# Autodesk Inventor assembly: Hooded Shooter MASTER
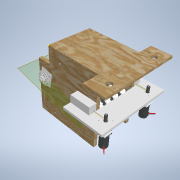
[picture p0: Inventor's stored thumbnail of the model, 180x180]
Saved by Autodesk Inventor 2020 (Build 240168000, 168)
## iProperties
Created: 2020-01-13
Part Number: Hooded Shooter MASTER
Document SubType Name: Assembly
Designer: autum
Author: autum
## Documents named in this file (17)
- D:\Users\JimAndVal\Documents\JIM\IronRiders\2020 Robot-1\Manipulators\Hooded Shooter (Protected Zone)\Hooded Shooter MASTER.iam
- D:\Users\JimAndVal\Documents\JIM\IronRiders\2020 Robot-1\Manipulators\Hooded Shooter (Protected Zone)\Hood.ipt
- D:\Users\JimAndVal\Documents\JIM\IronRiders\2020 Robot-1\Manipulators\Hooded Shooter (Protected Zone)\Hex Bearing.ipt
- D:\Users\JimAndVal\Documents\JIM\IronRiders\2020 Robot-1\Manipulators\Hooded Shooter (Protected Zone)\Hex Shaft.ipt
- D:\Users\JimAndVal\Documents\JIM\IronRiders\2020 Robot-1\Manipulators\Hooded Shooter (Protected Zone)\Hood (inside).ipt
- D:\Users\JimAndVal\Documents\JIM\IronRiders\2020 Robot-1\Manipulators\Hooded Shooter (Protected Zone)\Threaded rod.ipt
- D:\Users\JimAndVal\Documents\JIM\IronRiders\2020 Robot-1\Manipulators\Hooded Shooter (Protected Zone)\Shaft Mount with NEO mount.ipt
- D:\Users\JimAndVal\Documents\JIM\IronRiders\2020 Robot-1\Manipulators\Hooded Shooter (Protected Zone)\shooter bottom.ipt
- D:\Users\JimAndVal\Documents\JIM\IronRiders\2020 Robot-1\Manipulators\Hooded Shooter (Protected Zone)\am-2256 4 in HiGrip Wheel.iam
- D:\Users\JimAndVal\Documents\JIM\IronRiders\2020 Robot-1\Manipulators\Hooded Shooter (Protected Zone)\Shooter Base Cleat.ipt
- D:\Users\JimAndVal\Documents\JIM\IronRiders\2020 Robot-1\Manipulators\Hooded Shooter (Protected Zone)\1_5 inch PVC Spacer.ipt
- D:\Users\JimAndVal\Documents\JIM\IronRiders\2020 Robot-1\Manipulators\Hooded Shooter (Protected Zone)\Indexer Upper Plate.ipt
- D:\Users\JimAndVal\Documents\JIM\IronRiders\2020 Robot-1\Indexer 2.0\VersaPlanetary_v2_Single_Stage_10_1_with_BAG.iam
- D:\Users\JimAndVal\Documents\JIM\IronRiders\2020 Robot-1\Manipulators\Hooded Shooter (Protected Zone)\upper indexer plate cleat.ipt
- D:\Users\JimAndVal\Documents\JIM\IronRiders\2020 Robot-1\Manipulators\Hooded Shooter (Protected Zone)\Shooter Motor.iam
- D:\Users\JimAndVal\Documents\JIM\IronRiders\2020 Robot-1\Manipulators\Hooded Shooter (Protected Zone)\_16t_Aluminum_Hub_Sprocket_25_Chain_1_2_Hex_Bore_217-2642.ipt
- D:\Users\JimAndVal\Documents\JIM\IronRiders\2020 Robot-1\Manipulators\Hooded Shooter (Protected Zone)\Clamping_Shaft_Collar_-_1_2_Hex_ID_217-2737(1).ipt
## Components (39 placed, 16 different names)
1. Hood:1 — Mate:34, Flush:7, Mate:37, Mate:38, Mate:73, Mate:75
2. Hood:2 — Mate:35, Flush:6, Mate:40, Mate:72, Mate:74, Mate:79
3. Hex Bearing:1 — Mate:24, Mate:25, Insert:7
4. Hex Bearing:2 — Mate:14, Mate:15, Insert:8
5. Hex Shaft:1 — Mate:14, Mate:15, Mate:24, Mate:25, Flush:8, Mate:42, Mate:43, Mate:44, Mate:45, Mate:46, Mate:47, Mate:48, Mate:49, Mate:94, Flush:22
6. Hood (inside):1 — Mate:34, Mate:35, Flush:6, Flush:7, Mate:39, Mate:41, Mate:55, Mate:57, Mate:59, Mate:61, Mate:64, Mate:65
7. Threaded rod:2 — Mate:58, Mate:60, Mate:70, Mate:71, Mate:78
8. Threaded rod:3 — Mate:62, Mate:63, Mate:68, Mate:69, Mate:80
9. Threaded rod:4 — Mate:54, Mate:56, Mate:66, Mate:67, Mate:76
10. Shaft Mount with NEO mount:1 — Flush:1, Flush:2, Mate:33, Mate:36, Insert:8, Mate:53, Mate:76, Mate:78, Mate:80, Flush:10, Mate:88, Mate:92, Mate:93, Mate:96
11. Shaft Mount with NEO mount:2 — Flush:1, Flush:2, Flush:4, Mate:36, Mate:37, Mate:41, Insert:7, Flush:8, Mate:51, Mate:90
12. shooter bottom:1 — Mate:33, Flush:4, Mate:38, Mate:39, Mate:40, Mate:50, Mate:52, Flush:10, Flush:11, Flush:12, Flush:13, Flush:14, Mate:81
13. am-2256 4 in HiGrip Wheel:1 [sub-assembly] — Mate:42, Mate:43
14. am-2256 4 in HiGrip Wheel:2 [sub-assembly] — Mate:44, Mate:45
15. am-2256 4 in HiGrip Wheel:3 [sub-assembly] — Mate:48, Mate:49
16. am-2256 4 in HiGrip Wheel:4 [sub-assembly] — Mate:46, Mate:47
17. Shooter Base Cleat:1 — Mate:50, Mate:51, Flush:11, Flush:12
18. Shooter Base Cleat:2 — Mate:52, Mate:53
19. 1_5 inch PVC Spacer:1 — Mate:56, Mate:57
20. 1_5 inch PVC Spacer:2 — Mate:54, Mate:55
21. 1_5 inch PVC Spacer:3 — Mate:58, Mate:59
22. 1_5 inch PVC Spacer:4 — Mate:63, Mate:65
23. 1_5 inch PVC Spacer:5 — Mate:62, Mate:64
24. 1_5 inch PVC Spacer:6 — Mate:60, Mate:61
25. 1_5 inch PVC Spacer:7 — Mate:71, Mate:79
26. 1_5 inch PVC Spacer:8 — Mate:70
27. 1_5 inch PVC Spacer:9 — Mate:66, Mate:72
28. 1_5 inch PVC Spacer:10 — Mate:67, Mate:73
29. 1_5 inch PVC Spacer:11 — Mate:68, Mate:74
30. 1_5 inch PVC Spacer:12 — Mate:69, Mate:75
31. Indexer Upper Plate:1 — Flush:13, Flush:14, Mate:81, Mate:82, Mate:83, Mate:84, Flush:15, Flush:16, Mate:86, Mate:87, Angle:1, Flush:17, Mate:89, Flush:18, Mate:91
32. VersaPlanetary_v2_Single_Stage_10_1_with_BAG:1 [sub-assembly] — Mate:82, Mate:83, Mate:84, Mate:85
33. VersaPlanetary_v2_Single_Stage_10_1_with_BAG:2 [sub-assembly] — Mate:86, Mate:87, Angle:1
34. upper indexer plate cleat:1 — Mate:88, Flush:17, Mate:89
35. upper indexer plate cleat:2 — Mate:90, Flush:18, Mate:91
36. Shooter Motor:1 [sub-assembly] — Mate:92, Mate:93, Mate:95, Angle:2
37. _16t_Aluminum_Hub_Sprocket_25_Chain_1_2_Hex_Bore_217-2642:1 — Mate:97, Mate:98, Mate:99, Mate:100
38. Clamping_Shaft_Collar_-_1_2_Hex_ID_217-2737(1):1 — Mate:96, Mate:97, Mate:99, Flush:22
39. Clamping_Shaft_Collar_-_1_2_Hex_ID_217-2737(1):2 — Mate:98, Mate:100
## Relationships (92: Mate 71, Flush 17, Insert 2, Angle 2)
- Mate:14: Hex Bearing:2 ↔ Hex Shaft:1
- Mate:15: Hex Bearing:2 ↔ Hex Shaft:1
- Mate:24: Hex Bearing:1 ↔ Hex Shaft:1
- Mate:25: Hex Bearing:1 ↔ Hex Shaft:1
- Flush:1: Shaft Mount with NEO mount:1 ↔ Shaft Mount with NEO mount:2
- Flush:2: Shaft Mount with NEO mount:1 ↔ Shaft Mount with NEO mount:2
- Mate:33: Shaft Mount with NEO mount:1 ↔ shooter bottom:1
- Flush:4: Shaft Mount with NEO mount:2 ↔ shooter bottom:1
- Mate:34 (38.1 mm): Hood:1 ↔ Hood (inside):1
- Mate:35 (38.1 mm): Hood:2 ↔ Hood (inside):1
- Flush:6: Hood:2 ↔ Hood (inside):1
- Flush:7: Hood:1 ↔ Hood (inside):1
- Mate:36 (190.5 mm): Shaft Mount with NEO mount:1 ↔ Shaft Mount with NEO mount:2
- Mate:37 (38.1 mm): Hood:1 ↔ Shaft Mount with NEO mount:2
- Mate:38: Hood:1 ↔ shooter bottom:1
- Mate:39: Hood (inside):1 ↔ shooter bottom:1
- Mate:40: Hood:2 ↔ shooter bottom:1
- Mate:41: Hood (inside):1 ↔ Shaft Mount with NEO mount:2
- Insert:7: Hex Bearing:1 ↔ Shaft Mount with NEO mount:2
- Insert:8: Hex Bearing:2 ↔ Shaft Mount with NEO mount:1
- Flush:8 (-25.4 mm): Hex Shaft:1 ↔ Shaft Mount with NEO mount:2
- Mate:42: Hex Shaft:1 ↔ am-2256 4 in HiGrip Wheel:1
- Mate:43: Hex Shaft:1 ↔ am-2256 4 in HiGrip Wheel:1
- Mate:44: Hex Shaft:1 ↔ am-2256 4 in HiGrip Wheel:2
- Mate:45: Hex Shaft:1 ↔ am-2256 4 in HiGrip Wheel:2
- Mate:46: Hex Shaft:1 ↔ am-2256 4 in HiGrip Wheel:4
- Mate:47: Hex Shaft:1 ↔ am-2256 4 in HiGrip Wheel:4
- Mate:48: Hex Shaft:1 ↔ am-2256 4 in HiGrip Wheel:3
- Mate:49: Hex Shaft:1 ↔ am-2256 4 in HiGrip Wheel:3
- Mate:50: shooter bottom:1 ↔ Shooter Base Cleat:1
- Mate:51: Shaft Mount with NEO mount:2 ↔ Shooter Base Cleat:1
- Mate:52: shooter bottom:1 ↔ Shooter Base Cleat:2
- Mate:53: Shaft Mount with NEO mount:1 ↔ Shooter Base Cleat:2
- Mate:54: Threaded rod:4 ↔ 1_5 inch PVC Spacer:2
- Mate:55: Hood (inside):1 ↔ 1_5 inch PVC Spacer:2
- Mate:56: Threaded rod:4 ↔ 1_5 inch PVC Spacer:1
- Mate:57: Hood (inside):1 ↔ 1_5 inch PVC Spacer:1
- Mate:58: Threaded rod:2 ↔ 1_5 inch PVC Spacer:3
- Mate:59: Hood (inside):1 ↔ 1_5 inch PVC Spacer:3
- Mate:60: Threaded rod:2 ↔ 1_5 inch PVC Spacer:6
- Mate:61: Hood (inside):1 ↔ 1_5 inch PVC Spacer:6
- Mate:62: Threaded rod:3 ↔ 1_5 inch PVC Spacer:5
- Mate:63: Threaded rod:3 ↔ 1_5 inch PVC Spacer:4
- Mate:64: Hood (inside):1 ↔ 1_5 inch PVC Spacer:5
- Mate:65: Hood (inside):1 ↔ 1_5 inch PVC Spacer:4
- Mate:66: Threaded rod:4 ↔ 1_5 inch PVC Spacer:9
- Mate:67: Threaded rod:4 ↔ 1_5 inch PVC Spacer:10
- Mate:68: Threaded rod:3 ↔ 1_5 inch PVC Spacer:11
- Mate:69: Threaded rod:3 ↔ 1_5 inch PVC Spacer:12
- Mate:70: Threaded rod:2 ↔ 1_5 inch PVC Spacer:8
- Mate:71: Threaded rod:2 ↔ 1_5 inch PVC Spacer:7
- Mate:72: Hood:2 ↔ 1_5 inch PVC Spacer:9
- Mate:73: Hood:1 ↔ 1_5 inch PVC Spacer:10
- Mate:74: Hood:2 ↔ 1_5 inch PVC Spacer:11
- Mate:75: Hood:1 ↔ 1_5 inch PVC Spacer:12
- Mate:76: Threaded rod:4 ↔ Shaft Mount with NEO mount:1
- Mate:78: Threaded rod:2 ↔ Shaft Mount with NEO mount:1
- Mate:79: Hood:2 ↔ 1_5 inch PVC Spacer:7
- Mate:80: Threaded rod:3 ↔ Shaft Mount with NEO mount:1
- Flush:10: Shaft Mount with NEO mount:1 ↔ shooter bottom:1
- Flush:11: shooter bottom:1 ↔ Shooter Base Cleat:1
- Flush:12: shooter bottom:1 ↔ Shooter Base Cleat:1
- Flush:13: shooter bottom:1 ↔ Indexer Upper Plate:1
- Flush:14: shooter bottom:1 ↔ Indexer Upper Plate:1
- Mate:81 (165.1 mm): shooter bottom:1 ↔ Indexer Upper Plate:1
- Mate:82: Indexer Upper Plate:1 ↔ VersaPlanetary_v2_Single_Stage_10_1_with_BAG:1
- Mate:83: Indexer Upper Plate:1 ↔ VersaPlanetary_v2_Single_Stage_10_1_with_BAG:1
- Mate:84: Indexer Upper Plate:1 ↔ VersaPlanetary_v2_Single_Stage_10_1_with_BAG:1
- Flush:15 (-63.5 mm): Indexer Upper Plate:1
- Mate:85: VersaPlanetary_v2_Single_Stage_10_1_with_BAG:1
- Flush:16 (-63.5 mm): Indexer Upper Plate:1
- Mate:86: Indexer Upper Plate:1 ↔ VersaPlanetary_v2_Single_Stage_10_1_with_BAG:2
- Mate:87: Indexer Upper Plate:1 ↔ VersaPlanetary_v2_Single_Stage_10_1_with_BAG:2
- Angle:1 (180 deg): Indexer Upper Plate:1 ↔ VersaPlanetary_v2_Single_Stage_10_1_with_BAG:2
- Mate:88: Shaft Mount with NEO mount:1 ↔ upper indexer plate cleat:1
- Flush:17: Indexer Upper Plate:1 ↔ upper indexer plate cleat:1
- Mate:89: Indexer Upper Plate:1 ↔ upper indexer plate cleat:1
- Mate:90: Shaft Mount with NEO mount:2 ↔ upper indexer plate cleat:2
- Flush:18: Indexer Upper Plate:1 ↔ upper indexer plate cleat:2
- Mate:91: Indexer Upper Plate:1 ↔ upper indexer plate cleat:2
- Flush:21 (17.9578 mm)
- Mate:92: Shaft Mount with NEO mount:1 ↔ Shooter Motor:1
- Mate:93: Shaft Mount with NEO mount:1 ↔ Shooter Motor:1
- Mate:94: Hex Shaft:1
- Mate:95: Shooter Motor:1
- Angle:2 (90 deg): Shooter Motor:1
- Mate:96: Shaft Mount with NEO mount:1 ↔ Clamping_Shaft_Collar_-_1_2_Hex_ID_217-2737(1):1
- Mate:97: _16t_Aluminum_Hub_Sprocket_25_Chain_1_2_Hex_Bore_217-2642:1 ↔ Clamping_Shaft_Collar_-_1_2_Hex_ID_217-2737(1):1
- Mate:98: _16t_Aluminum_Hub_Sprocket_25_Chain_1_2_Hex_Bore_217-2642:1 ↔ Clamping_Shaft_Collar_-_1_2_Hex_ID_217-2737(1):2
- Mate:99: _16t_Aluminum_Hub_Sprocket_25_Chain_1_2_Hex_Bore_217-2642:1 ↔ Clamping_Shaft_Collar_-_1_2_Hex_ID_217-2737(1):1
- Mate:100: _16t_Aluminum_Hub_Sprocket_25_Chain_1_2_Hex_Bore_217-2642:1 ↔ Clamping_Shaft_Collar_-_1_2_Hex_ID_217-2737(1):2
- Flush:22: Hex Shaft:1 ↔ Clamping_Shaft_Collar_-_1_2_Hex_ID_217-2737(1):1
